# Autodesk Inventor assembly: assembly_truss
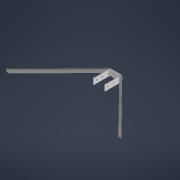
[picture p0: Inventor's stored thumbnail of the model, 180x180]
Saved by Autodesk Inventor 2021 (Build 250183000, 183)
## iProperties
Created: 2021-06-06
Part Number: assembly_truss
Document SubType Name: Assembly
Designer: Watchdog
Author: Watchdog
## Documents named in this file (4)
- C:\Users\Watchdog\OneDrive - Flinders\Advn Mech Design Shared\6_Development\2_Design\inventor\support\assembly_truss.iam
- C:\Users\Watchdog\OneDrive - Flinders\Advn Mech Design Shared\6_Development\2_Design\inventor\support\support_truss2.ipt
- C:\Users\Watchdog\OneDrive - Flinders\Advn Mech Design Shared\6_Development\2_Design\inventor\hoop_slider\hoop_tab_extender.ipt
- C:\Users\Watchdog\OneDrive - Flinders\Advn Mech Design Shared\6_Development\2_Design\inventor\support\trussSeparator.ipt
## Components (5 placed, 3 different names)
1. support_truss2:1 — Mate:1, Mate:6, Mate:7, Flush:1
2. support_truss2:2 — Mate:2, Mate:3, Mate:4, Mate:5, Flush:2, Flush:6
3. hoop_tab_extender:1 — Mate:4, Mate:5, Flush:2, Mate:8, Flush:5, Flush:7, Symmetry:1, Symmetry:2
4. hoop_tab_extender:2 — Mate:6, Mate:7, Flush:1, Mate:9, Flush:3, Flush:4, Symmetry:2
5. trussSeparator:1 — Mate:8, Mate:9, Flush:3, Flush:4, Flush:5
## Relationships (18: Mate 9, Flush 7, Symmetry 2)
- Mate:1: support_truss2:1
- Mate:2: support_truss2:2
- Mate:3: support_truss2:2
- Mate:4: support_truss2:2 ↔ hoop_tab_extender:1
- Mate:5: support_truss2:2 ↔ hoop_tab_extender:1
- Mate:6: support_truss2:1 ↔ hoop_tab_extender:2
- Mate:7: support_truss2:1 ↔ hoop_tab_extender:2
- Flush:1: support_truss2:1 ↔ hoop_tab_extender:2
- Flush:2: support_truss2:2 ↔ hoop_tab_extender:1
- Mate:8: hoop_tab_extender:1 ↔ trussSeparator:1
- Mate:9: hoop_tab_extender:2 ↔ trussSeparator:1
- Flush:3: hoop_tab_extender:2 ↔ trussSeparator:1
- Flush:4: hoop_tab_extender:2 ↔ trussSeparator:1
- Flush:5: hoop_tab_extender:1 ↔ trussSeparator:1
- Flush:6: support_truss2:2
- Flush:7: hoop_tab_extender:1
- Symmetry:1: hoop_tab_extender:1
- Symmetry:2: hoop_tab_extender:1 ↔ hoop_tab_extender:2
